# Autodesk Inventor assembly: A
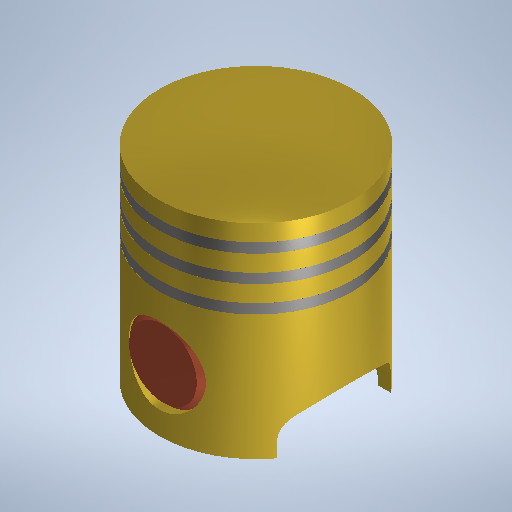
[picture p0: Inventor's stored thumbnail of the model, 512x512]
Saved by Autodesk Inventor 2025.2 (Build 292293000, 293)
## iProperties
Created: 2025-03-20
Part Number: A
Document SubType Name: Assembly
Designer: User
Author: User
## Documents named in this file (4)
- C:\Users\User\Documents\Inventor\Engine\A.iam
- C:\Users\User\Documents\Inventor\Engine\Part 1 Piston.ipt
- C:\Users\User\Documents\Inventor\Engine\Part 6 Pin.ipt
- C:\Users\User\Documents\Inventor\Engine\Part 5 Piston ring.ipt
## Components (5 placed, 3 different names)
1. Part 1 Piston:2 — Mate:1, Mate:2, Mate:3, Mate:4, Mate:5, Mate:6, Mate:7, Mate:8, Mate:9
2. Part 6 Pin:1 — Mate:7, Mate:8, Mate:9
3. Part 5 Piston ring:1 — Mate:1, Mate:4
4. Part 5 Piston ring:2 — Mate:2, Mate:5
5. Part 5 Piston ring:3 — Mate:3, Mate:6
## Relationships (9: Mate 9)
- Mate:1: Part 1 Piston:2 ↔ Part 5 Piston ring:1
- Mate:2: Part 1 Piston:2 ↔ Part 5 Piston ring:2
- Mate:3: Part 1 Piston:2 ↔ Part 5 Piston ring:3
- Mate:4: Part 1 Piston:2 ↔ Part 5 Piston ring:1
- Mate:5: Part 1 Piston:2 ↔ Part 5 Piston ring:2
- Mate:6: Part 1 Piston:2 ↔ Part 5 Piston ring:3
- Mate:7: Part 1 Piston:2 ↔ Part 6 Pin:1
- Mate:8: Part 1 Piston:2 ↔ Part 6 Pin:1
- Mate:9: Part 1 Piston:2 ↔ Part 6 Pin:1
